# Autodesk Inventor assembly: Actual Fucking Hindge
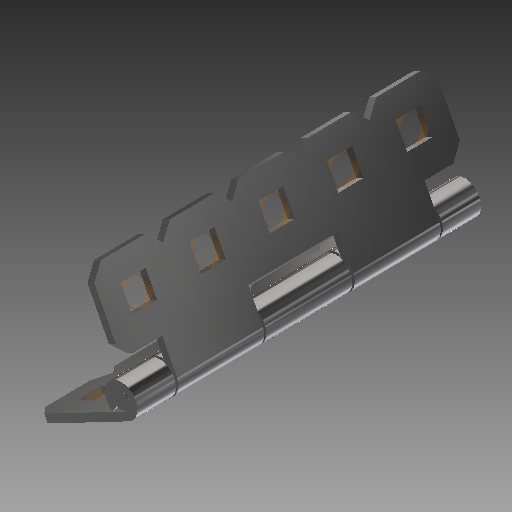
[picture p0: Inventor's stored thumbnail of the model, 512x512]
Saved by Autodesk Inventor 2019 (Build 230136000, 136)
## iProperties
Created: 2019-08-16
Part Number: Actual Fucking Hindge
Document SubType Name: Assembly
Designer: 43engineering
Author: 43engineering
## Documents named in this file (4)
- C:\Users\karlv\Documents\VEX\Karl CAD Lib\KarlCADLib\Gussets and Brackets\Actual Fucking Hindge.iam
- C:\Users\karlv\Documents\VEX\Karl CAD Lib\KarlCADLib\Gussets and Brackets\Hindge Pin.ipt
- C:\Users\karlv\Documents\VEX\Karl CAD Lib\KarlCADLib\Gussets and Brackets\Hindge Part.ipt
- C:\Users\karlv\Documents\VEX\Karl CAD Lib\KarlCADLib\Gussets and Brackets\Hindge Part B.ipt
## Components (3 placed, 3 different names)
1. Hindge Pin:1 — Mate:1, Flush:1, Mate:2
2. Hindge Part:1 — Mate:1, Flush:1, Flush:2
3. Hindge Part B:1 — Mate:2, Flush:2
## Relationships (4: Mate 2, Flush 2)
- Mate:1: Hindge Pin:1 ↔ Hindge Part:1
- Flush:1: Hindge Pin:1 ↔ Hindge Part:1
- Mate:2: Hindge Pin:1 ↔ Hindge Part B:1
- Flush:2: Hindge Part:1 ↔ Hindge Part B:1
